# Autodesk Inventor assembly: board
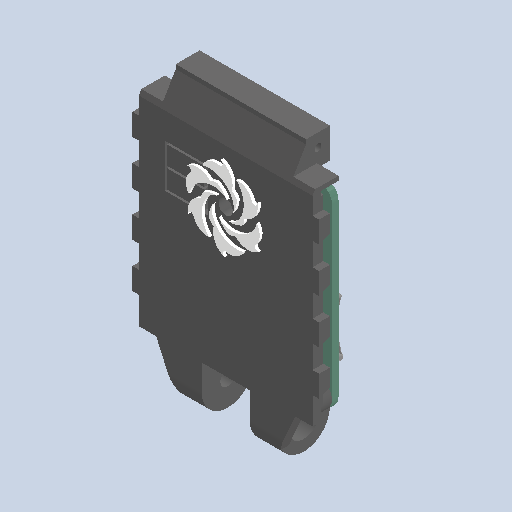
[picture p0: Inventor's stored thumbnail of the model, 512x512]
Saved by Autodesk Inventor 2026.1 (Build 301233020, 233B)
## iProperties
Created: 2026-01-21
Part Number: board
Document SubType Name: Assembly
Designer: hibik
Author: hibik
## Documents named in this file (4)
- C:\Users\hibik\Documents\Robomech\HR\Eglantyne_mark2\hard\board\board.iam
- C:\Users\hibik\Documents\Robomech\HR\Eglantyne_mark2\hard\board\protector.ipt
- C:\Users\hibik\Documents\Robomech\HR\Eglantyne_mark2\LOGO.ipt
- C:\Users\hibik\Documents\Robomech\HR\Eglantyne_mark2\hard\board\E-PIX.iam
## Components (3 placed, 3 different names)
1. protector:1 — フラッシュ:3, メイト:3, メイト:4, 挿入:1, 角度:1
2. LOGO:1 — フラッシュ:3, メイト:3, メイト:4
3. E-PIX:1 [sub-assembly] — 挿入:1, 角度:1
## Relationships (5: Mate 2, Flush 1, Insert 1, Angle 1)
- フラッシュ:3 [Flush]: protector:1 ↔ LOGO:1
- メイト:3 [Mate]: protector:1 ↔ LOGO:1
- メイト:4 [Mate] (11.28 mm): protector:1 ↔ LOGO:1
- 挿入:1 [Insert]: protector:1 ↔ E-PIX:1
- 角度:1 [Angle] (0 deg): protector:1 ↔ E-PIX:1
